# Autodesk Inventor assembly: Base Assembly
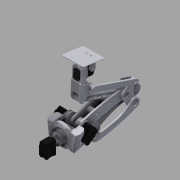
[picture p0: Inventor's stored thumbnail of the model, 180x180]
Saved by Autodesk Inventor 2017 (Build 210142000, 142)
## iProperties
Created: 2016-04-05
Part Number: Base Assembly
Document SubType Name: Assembly
Designer: alist
Author: alist
## Documents named in this file (37)
- F:\Documents\GitHub\EvoArm\Design\Assembly\Full.iam
- F:\Documents\GitHub\EvoArm\Design\Derived Parts\Base Plate.ipt
- F:\Documents\GitHub\EvoArm\Design\Derived Parts\Base Shaft.ipt
- F:\Documents\GitHub\EvoArm\Design\Derived Parts\Base Join.ipt
- F:\Documents\GitHub\EvoArm\Design\Parts\ax12_wheel.ipt
- F:\Documents\GitHub\EvoArm\Design\Arm - base center support.ipt
- F:\Documents\GitHub\EvoArm\Design\Arm - mounting top.ipt
- F:\Documents\GitHub\EvoArm\Design\Parts\ax12_box.ipt
- F:\Documents\GitHub\EvoArm\Design\Arm - mounting bottom.ipt
- F:\Documents\GitHub\EvoArm\Design\Arm - shoulder R.ipt
- F:\Documents\GitHub\EvoArm\Design\Arm - shoulder L.ipt
- F:\Documents\GitHub\EvoArm\Design\Arm - main arm L.ipt
- F:\Documents\GitHub\EvoArm\Design\Arm - main arm R.ipt
- F:\Documents\GitHub\EvoArm\Design\Arm - actuator hinge R.ipt
- F:\Documents\GitHub\EvoArm\Design\Arm - actuator hinge L.ipt
- F:\Documents\GitHub\EvoArm\Design\Arm - actuator linkage.ipt
- F:\Documents\GitHub\EvoArm\Design\Arm - parallel hinge.ipt
- F:\Documents\GitHub\EvoArm\Design\Arm - parallel linkage.ipt
- F:\Documents\GitHub\EvoArm\Design\Arm - stabilizer linkage.ipt
- F:\Documents\GitHub\EvoArm\Design\Arm - 608 bearing cap [Small].ipt
- F:\Documents\GitHub\EvoArm\Design\Parts\xl320_box.ipt
- F:\Documents\GitHub\EvoArm\Design\Parts\xl320_wheel.ipt
- F:\Documents\GitHub\EvoArm\Design\Arm - effector joint.ipt
- F:\Documents\GitHub\EvoArm\Design\Arm - effector hinge.ipt
- F:\Documents\GitHub\EvoArm\Design\Effector\Touchplate.ipt
- F:\Documents\GitHub\EvoArm\Design\DK2 Mount\Camera stand plate top.ipt
- F:\Documents\GitHub\EvoArm\Design\DK2 Mount\Camera mounting side.ipt
- F:\Documents\GitHub\EvoArm\Design\DK2 Mount\Camera mounting back.ipt
- F:\Documents\GitHub\EvoArm\Design\DK2 Mount\Camera stand plate base.ipt
- F:\Documents\GitHub\EvoArm\Design\DK2 Mount\Camera mount.ipt
- F:\Documents\GitHub\EvoArm\Design\DK2 Mount\Camera mount base bracing.ipt
- F:\Documents\GitHub\EvoArm\Design\DK2 Mount\Camera stabiliser.ipt
- F:\Documents\GitHub\EvoArm\Design\Parts\DK2 Camera.ipt
- F:\Documents\GitHub\EvoArm\Design\Arm - forearm v2.ipt
- F:\Documents\GitHub\EvoArm\Design\Arm - forearm v2 hinge.ipt
- F:\Documents\GitHub\EvoArm\Design\Arm - effector base v2.ipt
- F:\Documents\GitHub\EvoArm\Design\Arm - main arm spacer.ipt
## Components (45 placed, 36 different names)
1. Base Shaft:1 — Rigid:2, Rigid:5
2. Base Join:1 — Rigid:2, Rigid:3, Flush:1
3. ax12_wheel:1 — Rigid:3, Rotational:1
4. Arm - base center support:1 — Rigid:4, Rotational:4
5. Base Plate:3 — Rigid:4, Rigid:5, Rigid:10, Rigid:11
6. Arm - mounting top:1 — Flush:1, Rigid:6
7. ax12_box:1 — Rotational:1, Mate:1, Rigid:7
8. Arm - mounting bottom:1 — Rigid:6, Rigid:7, Flush:3, Rigid:21
9. Arm - shoulder R:1 — Rigid:9, Rigid:10
10. ax12_box:2 — Rigid:9, Rotational:2
11. ax12_wheel:2 — Rotational:2, Rigid:14
12. Arm - shoulder L:1 — Rigid:11, Rigid:12, Cylindrical:14, Flush:2
13. ax12_box:3 — Rigid:12, Rotational:3
14. ax12_wheel:3 — Rotational:3, Rigid:13
15. Arm - main arm L:1 — Rigid:13, Rigid:15, Rotational:12, Rigid:30, Rigid:31
16. Arm - main arm R:1 — Rigid:15, Rotational:17
17. Arm - actuator hinge R:1 — Rigid:14, Cylindrical:1
18. Arm - actuator hinge L:1 — Rotational:4, Rotational:6
19. Arm - actuator linkage:1 — Rotational:6, Cylindrical:1, Cylindrical:15
20. Arm - parallel hinge:1 — Rotational:12, Rotational:13, Rotational:16
21. Arm - parallel linkage:1 — Cylindrical:14, Rotational:13
22. Arm - stabilizer linkage:1 — Rotational:16, Cylindrical:16
23. Arm - 608 bearing cap [Small]:1 — Flush:2
24. xl320_box:1 — Rotational:14, Rigid:29
25. xl320_wheel:1 — Rotational:14, Rigid:17
26. Arm - effector joint:1 — Rigid:17, Rigid:18
27. xl320_box:2 — Rigid:18, Rotational:15
28. xl320_wheel:2 — Rotational:15, Rigid:19
29. Arm - effector hinge:1 — Rigid:19, Rigid:20
30. Touchplate:1 — Rigid:20
31. Camera stand plate top:1 — Flush:3, Rigid:21, Rigid:22, Rigid:23, Rigid:24, Flush:4
32. Camera mounting side:1 — Rigid:23, Rigid:25, Rigid:26
33. Camera mounting side:2 — Rigid:24
34. Camera mounting back:1 — Rigid:22, Flush:5
35. Camera stand plate base:1 — Flush:4
36. Camera mount:1 — Rigid:25, Flush:6
37. Camera mount base bracing:1 — Rigid:26
38. Camera stabiliser:1 — Flush:5
39. DK2 Camera:1 — Flush:6
40. Arm - forearm v2:1 — Rotational:17, Cylindrical:15, Rigid:27, Rigid:28
41. Arm - forearm v2 hinge:1 — Rigid:28
42. Arm - forearm v2 hinge:2 — Rigid:27, Rotational:18
43. Arm - effector base v2:1 — Rotational:18, Cylindrical:16, Rigid:29
44. Arm - main arm spacer:1 — Rigid:30
45. Arm - main arm spacer:2 — Rigid:31
## Relationships (52: WeldJoint 28, RevoluteJoint 12, Flush 6, CylindricalJoint 4, Mate 1, Angle 1)
- Rigid:2 [WeldJoint]: Base Shaft:1 ↔ Base Join:1
- Rigid:3 [WeldJoint]: Base Join:1 ↔ ax12_wheel:1
- Rigid:4 [WeldJoint]: Arm - base center support:1 ↔ Base Plate:3
- Rigid:5 [WeldJoint]: Base Shaft:1 ↔ Base Plate:3
- Flush:1: Base Join:1 ↔ Arm - mounting top:1
- Rotational:1 [RevoluteJoint]: ax12_wheel:1 ↔ ax12_box:1
- Mate:1: ax12_box:1
- Angle:1 (0 deg)
- Rigid:6 [WeldJoint]: Arm - mounting top:1 ↔ Arm - mounting bottom:1
- Rigid:7 [WeldJoint]: ax12_box:1 ↔ Arm - mounting bottom:1
- Rigid:9 [WeldJoint]: Arm - shoulder R:1 ↔ ax12_box:2
- Rotational:2 [RevoluteJoint]: ax12_box:2 ↔ ax12_wheel:2
- Rigid:10 [WeldJoint]: Base Plate:3 ↔ Arm - shoulder R:1
- Rigid:11 [WeldJoint]: Base Plate:3 ↔ Arm - shoulder L:1
- Rigid:12 [WeldJoint]: Arm - shoulder L:1 ↔ ax12_box:3
- Rotational:3 [RevoluteJoint]: ax12_box:3 ↔ ax12_wheel:3
- Rigid:13 [WeldJoint]: ax12_wheel:3 ↔ Arm - main arm L:1
- Rigid:14 [WeldJoint]: ax12_wheel:2 ↔ Arm - actuator hinge R:1
- Rotational:4 [RevoluteJoint]: Arm - base center support:1 ↔ Arm - actuator hinge L:1
- Rotational:6 [RevoluteJoint]: Arm - actuator hinge L:1 ↔ Arm - actuator linkage:1
- Cylindrical:1: Arm - actuator hinge R:1 ↔ Arm - actuator linkage:1
- Rigid:15 [WeldJoint] (23 mm): Arm - main arm L:1 ↔ Arm - main arm R:1
- Rotational:12 [RevoluteJoint] (-1 mm): Arm - main arm L:1 ↔ Arm - parallel hinge:1
- Cylindrical:14: Arm - shoulder L:1 ↔ Arm - parallel linkage:1
- Rotational:13 [RevoluteJoint] (1 mm): Arm - parallel hinge:1 ↔ Arm - parallel linkage:1
- Flush:2: Arm - shoulder L:1 ↔ Arm - 608 bearing cap [Small]:1
- Rotational:14 [RevoluteJoint]: xl320_box:1 ↔ xl320_wheel:1
- Rigid:17 [WeldJoint]: xl320_wheel:1 ↔ Arm - effector joint:1
- Rigid:18 [WeldJoint]: Arm - effector joint:1 ↔ xl320_box:2
- Rotational:15 [RevoluteJoint]: xl320_box:2 ↔ xl320_wheel:2
- Rigid:19 [WeldJoint]: xl320_wheel:2 ↔ Arm - effector hinge:1
- Rigid:20 [WeldJoint]: Arm - effector hinge:1 ↔ Touchplate:1
- Rotational:16 [RevoluteJoint] (-1 mm): Arm - parallel hinge:1 ↔ Arm - stabilizer linkage:1
- Flush:3: Arm - mounting bottom:1 ↔ Camera stand plate top:1
- Rigid:21 [WeldJoint]: Arm - mounting bottom:1 ↔ Camera stand plate top:1
- Rigid:22 [WeldJoint]: Camera stand plate top:1 ↔ Camera mounting back:1
- Rigid:23 [WeldJoint]: Camera stand plate top:1 ↔ Camera mounting side:1
- Rigid:24 [WeldJoint]: Camera stand plate top:1 ↔ Camera mounting side:2
- Flush:4: Camera stand plate top:1 ↔ Camera stand plate base:1
- Rigid:25 [WeldJoint]: Camera mounting side:1 ↔ Camera mount:1
- Rigid:26 [WeldJoint]: Camera mounting side:1 ↔ Camera mount base bracing:1
- Flush:5: Camera mounting back:1 ↔ Camera stabiliser:1
- Flush:6: Camera mount:1 ↔ DK2 Camera:1
- Rotational:17 [RevoluteJoint] (1 mm): Arm - main arm R:1 ↔ Arm - forearm v2:1
- Cylindrical:15: Arm - actuator linkage:1 ↔ Arm - forearm v2:1
- Rigid:27 [WeldJoint]: Arm - forearm v2:1 ↔ Arm - forearm v2 hinge:2
- Rigid:28 [WeldJoint]: Arm - forearm v2:1 ↔ Arm - forearm v2 hinge:1
- Rotational:18 [RevoluteJoint]: Arm - forearm v2 hinge:2 ↔ Arm - effector base v2:1
- Cylindrical:16: Arm - stabilizer linkage:1 ↔ Arm - effector base v2:1
- Rigid:29 [WeldJoint]: xl320_box:1 ↔ Arm - effector base v2:1
- Rigid:30 [WeldJoint]: Arm - main arm L:1 ↔ Arm - main arm spacer:1
- Rigid:31 [WeldJoint]: Arm - main arm L:1 ↔ Arm - main arm spacer:2
